# Autodesk Inventor assembly: Assembly1
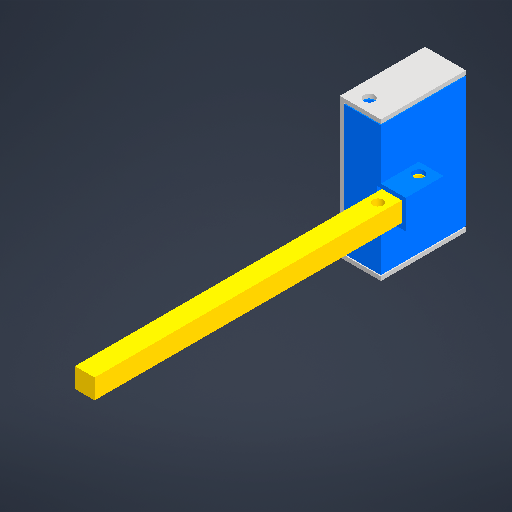
[picture p0: Inventor's stored thumbnail of the model, 512x512]
Saved by Autodesk Inventor 2026 (Build 300175000, 175)
## iProperties
Created: 2025-10-10
Part Number: Assembly1
Document SubType Name: Assembly
Designer: kenny
Author: kenny
## Documents named in this file (5)
- D:\Autodesk\Assembly1.iam
- D:\Users\kenny\Downloads\hc-sr04-ultrasonic-sensor-8.snapshot.15\hc-sr04\hc-sr04\hc-sr04.ipt
- D:\Autodesk\part\Part5.ipt
- D:\Autodesk\part\Part4.ipt
- D:\Autodesk\part\Part6.ipt
## Components (4 placed, 4 different names)
1. hc-sr04:1 — Mate:1, Mate:2
2. Part5:1 — Mate:1, Mate:2, Flush:1
3. Part4:1 — Flush:1, Flush:2
4. Part6:1 — Flush:2
## Relationships (4: Mate 2, Flush 2)
- Mate:1: hc-sr04:1 ↔ Part5:1
- Mate:2: hc-sr04:1 ↔ Part5:1
- Flush:1: Part5:1 ↔ Part4:1
- Flush:2: Part4:1 ↔ Part6:1
